# Autodesk Inventor assembly: llanta delantera
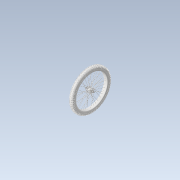
[picture p0: Inventor's stored thumbnail of the model, 180x180]
Saved by Autodesk Inventor 2021 (Build 250183000, 183)
## iProperties
Created: 2021-04-25
Part Number: llanta delantera
Document SubType Name: Assembly
Designer: j2seb
Author: j2seb
## Documents named in this file (4)
- C:\Git\Proyecto_APM\02 Inventor\llanta delantera.iam
- C:\Git\Proyecto_APM\02 Inventor\Ensamble_Llanta.iam
- C:\Git\Proyecto_APM\02 Inventor\eje_manzana_delantera.ipt
- C:\Users\j2seb\OneDrive\Documents\Inventor\Content Center Files\R2021\es-ES\DIN 6923\DIN 6923 - M10 x 1,5.ipt
## Components (4 placed, 3 different names)
1. Ensamble_Llanta:1 [sub-assembly] — Coincidencia:1, Coincidencia:2, Coincidencia:4
2. eje_manzana_delantera:1 — Coincidencia:1, Coincidencia:3, Coincidencia:5
3. DIN 6923 M10:1 — Coincidencia:3
4. DIN 6923 M10:2 — Coincidencia:5
## Relationships (5: Mate 5)
- Coincidencia:1 [Mate]: Ensamble_Llanta:1 ↔ eje_manzana_delantera:1
- Coincidencia:2 [Mate]: Ensamble_Llanta:1
- Coincidencia:3 [Mate]: eje_manzana_delantera:1 ↔ DIN 6923 M10:1
- Coincidencia:4 [Mate]: Ensamble_Llanta:1
- Coincidencia:5 [Mate]: eje_manzana_delantera:1 ↔ DIN 6923 M10:2
